# Autodesk Inventor assembly: Робот
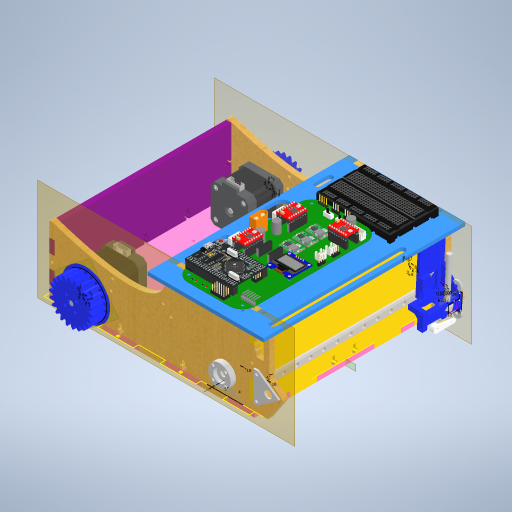
[picture p0: Inventor's stored thumbnail of the model, 512x512]
Saved by Autodesk Inventor 2024.2 (Build 282272000, 272)
## iProperties
Created: 2026-01-27
Part Number: Робот
Document SubType Name: Assembly
Designer: Service
d4: 0,000 мм
Author: Service
## Documents named in this file (17)
- C:\Users\Service\Documents\Artist-v2\3D\Робот.iam
- C:\Users\Service\Documents\Artist-v2\3D\Низ робота.ipt
- C:\Users\Service\Documents\Artist-v2\3D\бок.ipt
- C:\Users\Service\Documents\Artist-v2\3D\перед.ipt
- C:\Users\Service\Documents\Artist-v2\3D\NEMA17 42-40.ipt
- C:\Users\Service\Documents\Artist-v2\3D\Шестерня.ipt
- C:\Users\Service\Documents\Artist-v2\3D\stl\крепеж валика.ipt
- C:\Users\Service\Documents\Artist-v2\3D\dxf\спиралька.ipt
- C:\Users\Service\Documents\Artist-v2\3D\MGN7.ipt
- C:\Users\Service\Documents\Artist-v2\3D\stl\крышка.ipt
- C:\Users\Service\Documents\Artist-v2\3D\каретка.iam
- C:\Users\Service\Documents\Artist-v2\3D\Проект_ЕТЗ.iam
- C:\Users\Service\Documents\Artist-v2\3D\PROTOBOARD TOP.ipt
- C:\Users\Service\Documents\Artist-v2\3D\stl\задняя стенка.ipt
- C:\Users\Service\Documents\Artist-v2\3D\dxf\крепеж подшипника.ipt
- C:\Users\Service\Documents\Artist-v2\3D\stl\крепеж подшипника.ipt
- C:\Users\Service\Documents\Artist-v2\3D\stl\подшипник не выпадет.ipt
## Components (21 placed, 15 different names)
1. Низ робота:1 — Совмещение:2, Заподлицо:3, Совмещение:12, Заподлицо:9, Заподлицо:23, Заподлицо:25, Совмещение:47, Заподлицо:26, Заподлицо:27, Совмещение:58
2. бок:2 — Совмещение:2, Заподлицо:3, Совмещение:6, Совмещение:7, Совмещение:8, Совмещение:10, Совмещение:19, Совмещение:20, Заподлицо:21, Заподлицо:22, Совмещение:45, Заподлицо:24, Совмещение:48, Заподлицо:29, Совмещение:50, Совмещение:52, Совмещение:60, Заподлицо:32
3. перед:1 — Заподлицо:23, Заподлицо:24, Заподлицо:25, Совмещение:50, Совмещение:51, Заподлицо:30
4. NEMA17 42-40:1 — Совмещение:4, Совмещение:5, Совмещение:12, Совмещение:14
5. NEMA17 42-40:2 — Совмещение:6, Совмещение:7, Совмещение:8, Совмещение:9
6. Шестерня:1 — Совмещение:13, Совмещение:14
7. Шестерня:2 — Совмещение:42, Совмещение:43
8. Шестерня:3 — Совмещение:19, Совмещение:20
9. Шестерня:4 — Совмещение:9, Совмещение:10
10. крепеж валика:1 — Заподлицо:9
11. спиралька:1 — Заподлицо:21, Заподлицо:22, Совмещение:49
12. MGN7:1 — Совмещение:45, Совмещение:51, Заподлицо:30
13. крышка:1 — Совмещение:48, Заподлицо:29, Совмещение:55, Совмещение:56, Совмещение:57, Заподлицо:31
14. каретка:1 [sub-assembly] — Совмещение:49, Совмещение:52
15. Проект_ЕТЗ:1 [sub-assembly] — Совмещение:55, Совмещение:57
16. PROTOBOARD TOP:1 — Совмещение:56
17. задняя стенка:1 — Совмещение:58, Совмещение:59, Совмещение:60
18. крепеж подшипника:1 — Заподлицо:32
19. крепеж подшипника:2 — Заподлицо:33, Заподлицо:34, Заподлицо:36
20. подшипник не выпадет:1 — Заподлицо:35, Заподлицо:36
21. бок:1 — Совмещение:4, Совмещение:5, Совмещение:13, Совмещение:42, Совмещение:43, Совмещение:47, Заподлицо:26, Заподлицо:27, Заподлицо:31, Совмещение:59, Заподлицо:33, Заподлицо:34, Заподлицо:35
## Relationships (45: Mate 28, Flush 17)
- Совмещение:2 [Mate]: Низ робота:1 ↔ бок:2
- Заподлицо:3 [Flush]: Низ робота:1 ↔ бок:2
- Совмещение:4 [Mate]: NEMA17 42-40:1 ↔ бок:1
- Совмещение:5 [Mate]: NEMA17 42-40:1 ↔ бок:1
- Совмещение:6 [Mate]: бок:2 ↔ NEMA17 42-40:2
- Совмещение:7 [Mate]: бок:2 ↔ NEMA17 42-40:2
- Совмещение:8 [Mate]: бок:2 ↔ NEMA17 42-40:2
- Совмещение:9 [Mate]: NEMA17 42-40:2 ↔ Шестерня:4
- Совмещение:10 [Mate]: бок:2 ↔ Шестерня:4
- Совмещение:12 [Mate]: Низ робота:1 ↔ NEMA17 42-40:1
- Совмещение:13 [Mate]: Шестерня:1 ↔ бок:1
- Совмещение:14 [Mate]: NEMA17 42-40:1 ↔ Шестерня:1
- Совмещение:19 [Mate]: бок:2 ↔ Шестерня:3
- Совмещение:20 [Mate]: бок:2 ↔ Шестерня:3
- Заподлицо:9 [Flush]: Низ робота:1 ↔ крепеж валика:1
- Совмещение:42 [Mate]: Шестерня:2 ↔ бок:1
- Совмещение:43 [Mate]: Шестерня:2 ↔ бок:1
- Заподлицо:21 [Flush]: бок:2 ↔ спиралька:1
- Заподлицо:22 [Flush]: бок:2 ↔ спиралька:1
- Совмещение:45 [Mate]: бок:2 ↔ MGN7:1
- Заподлицо:23 [Flush]: Низ робота:1 ↔ перед:1
- Заподлицо:24 [Flush]: бок:2 ↔ перед:1
- Заподлицо:25 [Flush]: Низ робота:1 ↔ перед:1
- Совмещение:47 [Mate]: Низ робота:1 ↔ бок:1
- Заподлицо:26 [Flush]: Низ робота:1 ↔ бок:1
- Заподлицо:27 [Flush]: Низ робота:1 ↔ бок:1
- Совмещение:48 [Mate]: бок:2 ↔ крышка:1
- Заподлицо:29 [Flush]: бок:2 ↔ крышка:1
- Совмещение:49 [Mate]: спиралька:1 ↔ каретка:1
- Совмещение:50 [Mate]: бок:2 ↔ перед:1
- Совмещение:51 [Mate]: перед:1 ↔ MGN7:1
- Заподлицо:30 [Flush] (64.5 mm): перед:1 ↔ MGN7:1
- Совмещение:52 [Mate]: бок:2 ↔ каретка:1
- Совмещение:55 [Mate] (5 mm): крышка:1 ↔ Проект_ЕТЗ:1
- Совмещение:56 [Mate]: крышка:1 ↔ PROTOBOARD TOP:1
- Совмещение:57 [Mate]: крышка:1 ↔ Проект_ЕТЗ:1
- Заподлицо:31 [Flush]: крышка:1 ↔ бок:1
- Совмещение:58 [Mate]: Низ робота:1 ↔ задняя стенка:1
- Совмещение:59 [Mate]: задняя стенка:1 ↔ бок:1
- Совмещение:60 [Mate]: бок:2 ↔ задняя стенка:1
- Заподлицо:32 [Flush]: бок:2 ↔ крепеж подшипника:1
- Заподлицо:33 [Flush]: крепеж подшипника:2 ↔ бок:1
- Заподлицо:34 [Flush]: крепеж подшипника:2 ↔ бок:1
- Заподлицо:35 [Flush]: подшипник не выпадет:1 ↔ бок:1
- Заподлицо:36 [Flush]: крепеж подшипника:2 ↔ подшипник не выпадет:1
